# Autodesk Inventor assembly: OdroidAssembly
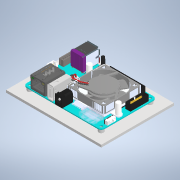
[picture p0: Inventor's stored thumbnail of the model, 180x180]
Saved by Autodesk Inventor 2020 (Build 240168000, 168)
## iProperties
Created: 2019-06-15
Part Number: OdroidAssembly
Document SubType Name: Assembly
Designer: amirt
Author: amirt
## Documents named in this file (6)
- C:\Users\amirt\Documents\Inventor\Drone\OdroidAssembly.iam
- C:\Users\amirt\Documents\Inventor\Drone\Imported Components\Odroid-XU4 v1.ipt
- C:\Users\amirt\Documents\Inventor\Drone\3DPrint\odroidstandoff.ipt
- C:\Users\amirt\Documents\Inventor\Drone\3DPrint\BasePlate.ipt
- C:\Users\amirt\Documents\Inventor\Drone\Imported Components\PM04_V1.ipt
- C:\Users\amirt\Documents\Inventor\Drone\Imported Components\PM04_V2.ipt
## Components (8 placed, 5 different names)
1. Odroid-XU4 v1:1 — Flush:1, Flush:2, Mate:1, Insert:1, Mate:2, Mate:3
2. odroidstandoff:1 — Flush:1, Flush:2
3. odroidstandoff:2 — Mate:2
4. odroidstandoff:3 — Mate:1, Insert:1
5. odroidstandoff:4 — Mate:3
6. BasePlate:1 — Flush:3, Mate:4, Mate:5, Flush:4, Flush:5, Flush:6
7. PM04_V1:1 — Flush:3, Mate:4, Flush:6
8. PM04_V2:1 — Mate:5, Flush:4, Flush:5
## Relationships (12: Flush 6, Mate 5, Insert 1)
- Flush:1: Odroid-XU4 v1:1 ↔ odroidstandoff:1
- Flush:2: Odroid-XU4 v1:1 ↔ odroidstandoff:1
- Mate:1: Odroid-XU4 v1:1 ↔ odroidstandoff:3
- Insert:1: Odroid-XU4 v1:1 ↔ odroidstandoff:3
- Mate:2: Odroid-XU4 v1:1 ↔ odroidstandoff:2
- Mate:3: Odroid-XU4 v1:1 ↔ odroidstandoff:4
- Flush:3 (13.7033 mm): BasePlate:1 ↔ PM04_V1:1
- Mate:4: BasePlate:1 ↔ PM04_V1:1
- Mate:5: BasePlate:1 ↔ PM04_V2:1
- Flush:4 (24.7015 mm): BasePlate:1 ↔ PM04_V2:1
- Flush:5 (15.8242 mm): BasePlate:1 ↔ PM04_V2:1
- Flush:6 (9.7917 mm): BasePlate:1 ↔ PM04_V1:1
